# Autodesk Inventor assembly: 組合1
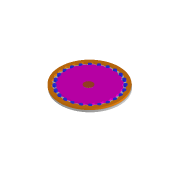
[picture p0: Inventor's stored thumbnail of the model, 180x180]
Saved by Autodesk Inventor 2022 (Build 260153000, 153)
## iProperties
Created: 2023-11-18
Part Number: 組合1
Document SubType Name: Assembly
Designer: JOU
Author: JOU
## Documents named in this file (6)
- C:\Users\JOU\Desktop\git\Special-project\Cycloidal Gear\inventor\double\組合1.iam
- C:\Users\JOU\Desktop\git\Special-project\Cycloidal Gear\inventor\double\hypocycloid.ipt
- C:\Users\JOU\Desktop\git\Special-project\Cycloidal Gear\inventor\double\epicycloid.ipt
- C:\Users\JOU\Desktop\git\Special-project\Cycloidal Gear\inventor\double\pin.ipt
- C:\Users\JOU\Desktop\git\Special-project\Cycloidal Gear\inventor\double\input.ipt
- C:\Users\JOU\Desktop\git\Special-project\Cycloidal Gear\inventor\double\pindisk.ipt
## Components (28 placed, 5 different names)
1. hypocycloid:1 — 齊平:27, 相切:1, 相切:2, 齊平:28, 貼合:31
2. epicycloid:1 — 齊平:3, 貼合:1, 齊平:28
3. input:1 — 齊平:3, 貼合:1, 角度:1, 貼合:31
4. pindisk:1 — 貼合:2, 貼合:3, 貼合:4, 貼合:5, 貼合:6, 貼合:7, 貼合:8, 貼合:9, 貼合:10, 貼合:11, 貼合:12, 貼合:13, 貼合:14, 貼合:15, 貼合:16, 貼合:17, 貼合:18, 貼合:19, 貼合:20, 貼合:21, 貼合:22, 貼合:23, 貼合:24, 貼合:25, 貼合:26, 貼合:27, 貼合:28, 貼合:29, 貼合:30
5. pin:2 — 貼合:2, 齊平:4, 貼合:3, 貼合:27
6. pin:3 — 齊平:4, 齊平:5, 貼合:4, 貼合:28
7. pin:4 — 齊平:5, 齊平:6, 貼合:5, 貼合:29
8. pin:5 — 齊平:6, 齊平:7, 貼合:6
9. pin:6 — 齊平:7, 齊平:8, 貼合:7, 相切:2
10. pin:7 — 齊平:8, 齊平:9, 貼合:8, 相切:1
11. pin:8 — 齊平:9, 齊平:10, 貼合:9, 貼合:30
12. pin:9 — 齊平:10, 齊平:11, 貼合:10
13. pin:10 — 齊平:11, 齊平:12, 貼合:11
14. pin:11 — 齊平:12, 齊平:13, 貼合:12
15. pin:12 — 齊平:13, 齊平:14, 貼合:13, 齊平:27
16. pin:13 — 齊平:14, 齊平:15, 貼合:14
17. pin:14 — 齊平:15, 齊平:16, 貼合:15
18. pin:15 — 齊平:16, 齊平:17, 貼合:16
19. pin:16 — 齊平:17, 齊平:18, 貼合:17
20. pin:17 — 齊平:18, 齊平:19, 貼合:18
21. pin:18 — 齊平:19, 齊平:20, 貼合:19
22. pin:19 — 齊平:20, 齊平:21, 貼合:20
23. pin:20 — 齊平:21, 齊平:22, 貼合:21
24. pin:21 — 齊平:22, 齊平:23, 貼合:22
25. pin:22 — 齊平:23, 齊平:24, 貼合:23
26. pin:23 — 齊平:24, 齊平:25, 貼合:24
27. pin:24 — 齊平:25, 齊平:26, 貼合:25
28. pin:25 — 齊平:26, 貼合:26
## Relationships (60: Mate 31, Flush 26, Tangent 2, Angle 1)
- 齊平:3 [Flush]: epicycloid:1 ↔ input:1
- 貼合:1 [Mate]: epicycloid:1 ↔ input:1
- 貼合:2 [Mate]: pindisk:1 ↔ pin:2
- 齊平:4 [Flush]: pin:2 ↔ pin:3
- 齊平:5 [Flush]: pin:3 ↔ pin:4
- 齊平:6 [Flush]: pin:4 ↔ pin:5
- 齊平:7 [Flush]: pin:5 ↔ pin:6
- 齊平:8 [Flush]: pin:6 ↔ pin:7
- 齊平:9 [Flush]: pin:7 ↔ pin:8
- 齊平:10 [Flush]: pin:8 ↔ pin:9
- 齊平:11 [Flush]: pin:9 ↔ pin:10
- 齊平:12 [Flush]: pin:10 ↔ pin:11
- 齊平:13 [Flush]: pin:11 ↔ pin:12
- 齊平:14 [Flush]: pin:12 ↔ pin:13
- 齊平:15 [Flush]: pin:13 ↔ pin:14
- 齊平:16 [Flush]: pin:14 ↔ pin:15
- 齊平:17 [Flush]: pin:15 ↔ pin:16
- 齊平:18 [Flush]: pin:16 ↔ pin:17
- 齊平:19 [Flush]: pin:17 ↔ pin:18
- 齊平:20 [Flush]: pin:18 ↔ pin:19
- 齊平:21 [Flush]: pin:19 ↔ pin:20
- 齊平:22 [Flush]: pin:20 ↔ pin:21
- 齊平:23 [Flush]: pin:21 ↔ pin:22
- 齊平:24 [Flush]: pin:22 ↔ pin:23
- 齊平:25 [Flush]: pin:23 ↔ pin:24
- 齊平:26 [Flush]: pin:24 ↔ pin:25
- 貼合:3 [Mate]: pindisk:1 ↔ pin:2
- 貼合:4 [Mate]: pindisk:1 ↔ pin:3
- 貼合:5 [Mate]: pindisk:1 ↔ pin:4
- 貼合:6 [Mate]: pindisk:1 ↔ pin:5
- 貼合:7 [Mate]: pindisk:1 ↔ pin:6
- 貼合:8 [Mate]: pindisk:1 ↔ pin:7
- 貼合:9 [Mate]: pindisk:1 ↔ pin:8
- 貼合:10 [Mate]: pindisk:1 ↔ pin:9
- 貼合:11 [Mate]: pindisk:1 ↔ pin:10
- 貼合:12 [Mate]: pindisk:1 ↔ pin:11
- 貼合:13 [Mate]: pindisk:1 ↔ pin:12
- 貼合:14 [Mate]: pindisk:1 ↔ pin:13
- 貼合:15 [Mate]: pindisk:1 ↔ pin:14
- 貼合:16 [Mate]: pindisk:1 ↔ pin:15
- 貼合:17 [Mate]: pindisk:1 ↔ pin:16
- 貼合:18 [Mate]: pindisk:1 ↔ pin:17
- 貼合:19 [Mate]: pindisk:1 ↔ pin:18
- 貼合:20 [Mate]: pindisk:1 ↔ pin:19
- 貼合:21 [Mate]: pindisk:1 ↔ pin:20
- 貼合:22 [Mate]: pindisk:1 ↔ pin:21
- 貼合:23 [Mate]: pindisk:1 ↔ pin:22
- 貼合:24 [Mate]: pindisk:1 ↔ pin:23
- 貼合:25 [Mate]: pindisk:1 ↔ pin:24
- 貼合:26 [Mate]: pindisk:1 ↔ pin:25
- 貼合:27 [Mate]: pindisk:1 ↔ pin:2
- 貼合:28 [Mate]: pindisk:1 ↔ pin:3
- 貼合:29 [Mate]: pindisk:1 ↔ pin:4
- 貼合:30 [Mate]: pindisk:1 ↔ pin:8
- 齊平:27 [Flush]: hypocycloid:1 ↔ pin:12
- 相切:1 [Tangent]: hypocycloid:1 ↔ pin:7
- 相切:2 [Tangent]: hypocycloid:1 ↔ pin:6
- 齊平:28 [Flush]: hypocycloid:1 ↔ epicycloid:1
- 角度:1 [Angle] (0 deg): input:1
- 貼合:31 [Mate]: hypocycloid:1 ↔ input:1
